# Autodesk Inventor assembly: RelicArmLance
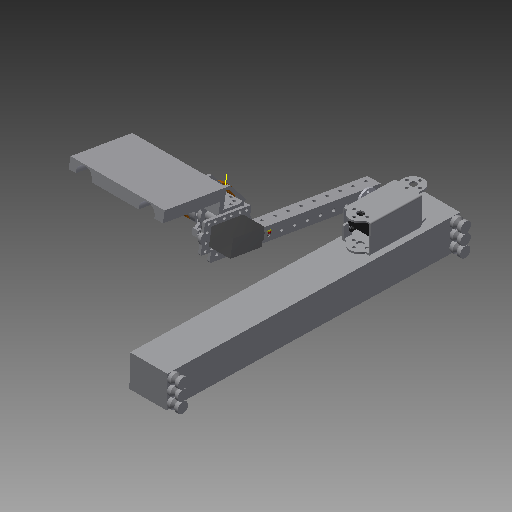
[picture p0: Inventor's stored thumbnail of the model, 512x512]
Saved by Autodesk Inventor 2017 (Build 210142000, 142)
## iProperties
Created: 2018-02-16
Part Number: RelicArmLance
Document SubType Name: Assembly
Designer: User
Author: User
## Documents named in this file (8)
- C:\Robotics\CAD\2017-18_CAD\RelicArmLance.iam
- C:\Robotics\CAD\2016-17_CAD\Lift2.iam
- C:\Robotics\CAD\COTSParts\Tetrix\39197_txm-485hb standard servo with horn.ipt
- C:\Robotics\CAD\COTSParts\Tetrix\ptp_tetrix_servoframe_bracket.ipt
- C:\Robotics\CAD\COTSParts\Tetrix\Tetrix angle 208mm.ipt
- C:\Robotics\CAD\COTSParts\Tetrix\Servo with servo blocks.ipt
- C:\Robotics\CAD\2017-18_CAD\claw beta.ipt
- C:\Robotics\CAD\2017-18_CAD\relicmold.ipt
## Components (7 placed, 7 different names)
1. Lift2:1 [sub-assembly] — Mate:4, Flush:1, Flush:2
2. 39197_txm-485hb standard servo with horn:1 — Mate:1, Mate:2, Mate:3, Flush:1, Mate:42, Mate:43, Mate:44
3. ptp_tetrix_servoframe_bracket:1 — Mate:1, Mate:2, Mate:3, Mate:4, Flush:2
4. Tetrix angle 208mm:1 — Mate:9, Mate:10, Angle:1, Mate:42, Mate:43, Mate:44
5. Servo with servo blocks:1 — Mate:9, Mate:10, Angle:1, Mate:47, Mate:48, Mate:49, Mate:50, Mate:51
6. claw beta:1 — Mate:48, Mate:49
7. relicmold:1 — Mate:47, Mate:50, Mate:51
## Relationships (17: Mate 14, Flush 2, Angle 1)
- Mate:1: 39197_txm-485hb standard servo with horn:1 ↔ ptp_tetrix_servoframe_bracket:1
- Mate:2: 39197_txm-485hb standard servo with horn:1 ↔ ptp_tetrix_servoframe_bracket:1
- Mate:3: 39197_txm-485hb standard servo with horn:1 ↔ ptp_tetrix_servoframe_bracket:1
- Mate:4: Lift2:1 ↔ ptp_tetrix_servoframe_bracket:1
- Flush:1 (50.8 mm): Lift2:1 ↔ 39197_txm-485hb standard servo with horn:1
- Flush:2 (6.35 mm): Lift2:1 ↔ ptp_tetrix_servoframe_bracket:1
- Mate:9: Tetrix angle 208mm:1 ↔ Servo with servo blocks:1
- Mate:10: Tetrix angle 208mm:1 ↔ Servo with servo blocks:1
- Angle:1 (0 deg): Tetrix angle 208mm:1 ↔ Servo with servo blocks:1
- Mate:42 (8.001 mm): 39197_txm-485hb standard servo with horn:1 ↔ Tetrix angle 208mm:1
- Mate:43 (8.001 mm): 39197_txm-485hb standard servo with horn:1 ↔ Tetrix angle 208mm:1
- Mate:44: 39197_txm-485hb standard servo with horn:1 ↔ Tetrix angle 208mm:1
- Mate:47: Servo with servo blocks:1 ↔ relicmold:1
- Mate:48: Servo with servo blocks:1 ↔ claw beta:1
- Mate:49: Servo with servo blocks:1 ↔ claw beta:1
- Mate:50: Servo with servo blocks:1 ↔ relicmold:1
- Mate:51: Servo with servo blocks:1 ↔ relicmold:1
